# Autodesk Inventor assembly: LR_06
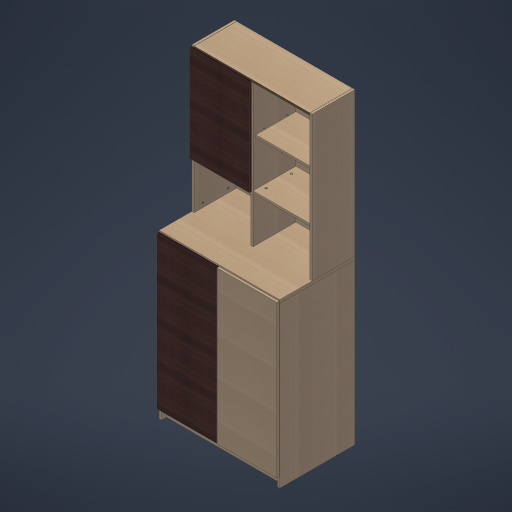
[picture p0: Inventor's stored thumbnail of the model, 512x512]
Saved by Autodesk Inventor 2024.3 (Build 283343000, 343)
## iProperties
Created: 2013-04-02
Part Number: LR_06
Document SubType Name: Assembly
Designer: User
Description: Side Shelf
Author: User
## Documents named in this file (30)
- C:\W4INV 2024 Design\PROJECTS\Living Room\Side Cabinet\LR_06.iam
- C:\W4INV 2024 Design\PROJECTS\Samples\Living Room\Side Cabinet\LR_0604.ipt
- C:\W4INV 2024 Design\PROJECTS\Samples\Living Room\Side Cabinet\LR_0611.ipt
- C:\W4INV 2024 Design\PROJECTS\Samples\Living Room\Side Cabinet\LR_0605.ipt
- C:\W4INV 2024 Design\PROJECTS\Samples\Living Room\Side Cabinet\LR_0608.ipt
- C:\W4INV 2024 Design\PROJECTS\Samples\Living Room\Side Cabinet\LR_0613.ipt
- C:\W4INV 2024 Design\PROJECTS\Samples\Living Room\Side Cabinet\LR_0607.ipt
- C:\W4INV 2024 Design\PROJECTS\Samples\Living Room\Side Cabinet\LR_0612.ipt
- C:\W4INV 2024 Design\PROJECTS\Samples\Living Room\Side Cabinet\LR_0606.ipt
- C:\W4INV 2024 Design\PROJECTS\Samples\Living Room\Side Cabinet\LR_0617.ipt
- C:\W4INV 2024 Design\PROJECTS\Samples\Living Room\Side Cabinet\LR_0616.ipt
- C:\W4INV 2024 Design\PROJECTS\Samples\Living Room\Side Cabinet\LR_0610.ipt
- C:\W4INV 2024 Design\PROJECTS\Samples\Living Room\Side Cabinet\LR_0609.ipt
- C:\W4INV 2024 Design\PROJECTS\Samples\Living Room\Side Cabinet\LR_0614.ipt
- C:\W4INV 2024 Design\PROJECTS\Samples\Living Room\Side Cabinet\LR_0619.ipt
- C:\W4INV 2024 Design\PROJECTS\Samples\Living Room\Side Cabinet\LR_0602.ipt
- C:\W4INV 2024 Design\PROJECTS\Samples\Living Room\Side Cabinet\LR_0618.ipt
- C:\W4INV 2024 Design\PROJECTS\Samples\Living Room\Side Cabinet\LR_0615.ipt
- C:\W4INV 2024 Design\PROJECTS\Samples\Living Room\Side Cabinet\SkeletonLR_0600.ipt
- C:\W4INV 2024 Design\PROJECTS\Samples\Living Room\Side Cabinet\LR_0601.ipt
- C:\W4INV 2024 Design\PROJECTS\Samples\Living Room\Side Cabinet\LR_0603.ipt
- C:\W4INV 2024 Design\_LIBRARY\Hinges\CONCEALED HINGE\Full Overlay Hinge Wood Screw Cup Wood Screw T18.iam
- C:\W4INV 2024 Design\_LIBRARY\Holders\Shelf holder D5\Shelf support D5 L16 HOL 3 CAP ON.ipt
- C:\W4INV 2024 Design\_LIBRARY\Fixed joints\Minifix joint\MINIFIX D15 v2\Minifix D15 & Dowel L34 & Cap D15 PB T18 LH.ipt
- C:\W4INV 2024 Design\_LIBRARY\Fixed joints\Minifix joint\MINIFIX D15 v2\Minifix D15 & Dowel L34 & Cap D15 PB T18 RH.ipt
- C:\W4INV 2024 Design\_LIBRARY\Supports and legs\Supports\ADJUSTABLE SUPPORT\Support M6 H27 D18 with Bushing SB T18.ipt
- C:\W4INV 2023 Design\LIBRARY\Hinges\CONCEALED HINGE.iam
- C:\W4INV 2023 Design\LIBRARY\Holders\Shelf holder D5.ipt
- C:\W4INV 2023 Design\LIBRARY\Supports and legs\Supports\ADJUSTABLE SUPPORT.ipt
- C:\W4INV 2023 Design\LIBRARY\Fixed joints\Minifix joint\MINIFIX D15 v2.ipt
## Components (84 placed, 24 different names)
1. LR_0604-Top Partition:1 — Mate:98, Mate:100, Mate:102, Mate:104, Mate:106, Mate:108, Mate:114, Mate:118, Mate:138, Mate:140, Mate:142, Mate:144
2. LR_0611-Left Side:1 — Flush:7, Flush:8, Mate:32, Flush:107, Mate:34, Flush:108, Mate:44, Mate:50, Flush:113, Mate:84, Mate:86, Flush:115, Mate:88, Mate:90, Mate:122, Mate:126, Flush:143, Flush:145
3. LR_0605-Right Side:1 — Mate:40, Flush:111, Mate:42, Flush:112, Flush:114, Flush:116, Mate:124, Mate:128, Flush:144, Flush:146
4. LR_0608-Bottom:1 — Mate:116, Mate:120, Flush:135, Flush:136, Flush:137, Flush:138
5. LR_0613-Left Door:1 — Flush:3, Flush:4
6. LR_0607-Right Door:1
7. LR_0612-Left Upper Side:1 — Flush:5, Flush:6, Mate:36, Flush:109, Mate:38, Flush:110, Mate:56, Mate:68, Flush:123, Flush:126, Mate:130, Mate:134, Mate:146, Mate:154
8. LR_0606-Right Upper Side:1 — Mate:65, Mate:77, Flush:124, Flush:127, Mate:132, Mate:136, Mate:152, Mate:160
9. LR_0617-Top:1 — Mate:110, Mate:112, Flush:139, Flush:140, Flush:141, Flush:142
10. LR_0616-Vertical Upper Partition:1 — Mate:59, Mate:62, Mate:71, Mate:74, Flush:125, Flush:128, Flush:129, Flush:130, Mate:148, Mate:150, Mate:156, Mate:158
11. LR_0610-Left Horizontal Partition:1 — Flush:147, Flush:148, Flush:149, Flush:150, Flush:151, Flush:152, Flush:153, Flush:154
12. LR_0609-Right Horizontal Partition:1
13. LR_0619-Upper Door:1 — Flush:1, Flush:2
14. LR_0602-Lower Back:1
15. LR_0618-Top Back:1
16. LR_0615-Plynth:1
17. LR_0603-Lover Vertical Partition:1 — Mate:47, Mate:53, Flush:131, Flush:132, Flush:133, Flush:134
18. Full Overlay Hinge Wood Screw Cup Wood Screw T18:1 [sub-assembly] — Mate:31, Mate:32, Flush:107
19. Full Overlay Hinge Wood Screw Cup Wood Screw T18:2 [sub-assembly] — Mate:33, Mate:34, Flush:108
20. Full Overlay Hinge Wood Screw Cup Wood Screw T18:3 [sub-assembly] — Mate:35, Mate:36, Flush:109
21. Full Overlay Hinge Wood Screw Cup Wood Screw T18:4 [sub-assembly] — Mate:37, Mate:38, Flush:110
22. Full Overlay Hinge Wood Screw Cup Wood Screw T18:5 [sub-assembly] — Mate:39, Mate:40, Flush:111
23. Full Overlay Hinge Wood Screw Cup Wood Screw T18:6 [sub-assembly] — Mate:41, Mate:42, Flush:112
24. Shelf support D5 L16 HOL 3 CAP ON:13 — Mate:56, Mate:57, Mate:79
25. Shelf support D5 L16 HOL 3 CAP ON:14 — Mate:59, Mate:60, Mate:80
26. Shelf support D5 L16 HOL 3 CAP ON:15 — Mate:62, Mate:63, Mate:81
27. Shelf support D5 L16 HOL 3 CAP ON:16 — Mate:65, Mate:66, Mate:82
28. Shelf support D5 L16 HOL 3 CAP ON:17 — Mate:67, Mate:68, Mate:69
29. Shelf support D5 L16 HOL 3 CAP ON:18 — Mate:70, Mate:71, Mate:72
30. Shelf support D5 L16 HOL 3 CAP ON:19 — Mate:73, Mate:74, Mate:75
31. Shelf support D5 L16 HOL 3 CAP ON:20 — Mate:76, Mate:77, Mate:78
32. Support M6 H27 D18 with Bushing SB T18:6 — Mate:83, Flush:113, Mate:84
33. Support M6 H27 D18 with Bushing SB T18:7 — Mate:85, Flush:114, Mate:86
34. Support M6 H27 D18 with Bushing SB T18:8 — Mate:87, Flush:115, Mate:88
35. Support M6 H27 D18 with Bushing SB T18:9 — Mate:89, Flush:116, Mate:90
36. Minifix D15 & Dowel L34 & Cap D15 PB T18 RH:7 — Mate:97, Flush:123, Mate:98
37. Minifix D15 & Dowel L34 & Cap D15 PB T18 LH:8 — Mate:99, Flush:124, Mate:100
38. Minifix D15 & Dowel L34 & Cap D15 PB T18 LH:9 — Mate:101, Flush:125, Mate:102
39. Minifix D15 & Dowel L34 & Cap D15 PB T18 LH:10 — Mate:103, Flush:126, Mate:104
40. Minifix D15 & Dowel L34 & Cap D15 PB T18 RH:11 — Mate:105, Flush:127, Mate:106
41. Minifix D15 & Dowel L34 & Cap D15 PB T18 RH:12 — Mate:107, Flush:128, Mate:108
42. Minifix D15 & Dowel L34 & Cap D15 PB T18 RH:13 — Mate:109, Mate:110, Flush:129
43. Minifix D15 & Dowel L34 & Cap D15 PB T18 LH:14 — Mate:111, Mate:112, Flush:130
44. Minifix D15 & Dowel L34 & Cap D15 PB T18 RH:15 — Mate:113, Mate:114, Flush:131
45. Minifix D15 & Dowel L34 & Cap D15 PB T18 LH:16 — Mate:115, Mate:116, Flush:132
46. Minifix D15 & Dowel L34 & Cap D15 PB T18 LH:17 — Mate:117, Mate:118, Flush:133
47. Minifix D15 & Dowel L34 & Cap D15 PB T18 RH:18 — Mate:119, Mate:120, Flush:134
48. Minifix D15 & Dowel L34 & Cap D15 PB T18 LH:19 — Mate:121, Mate:122, Flush:135
49. Minifix D15 & Dowel L34 & Cap D15 PB T18 RH:20 — Mate:123, Mate:124, Flush:136
50. Minifix D15 & Dowel L34 & Cap D15 PB T18 RH:21 — Mate:125, Mate:126, Flush:137
51. Minifix D15 & Dowel L34 & Cap D15 PB T18 LH:22 — Mate:127, Mate:128, Flush:138
52. Minifix D15 & Dowel L34 & Cap D15 PB T18 RH:23 — Mate:129, Mate:130, Flush:139
53. Minifix D15 & Dowel L34 & Cap D15 PB T18 LH:24 — Mate:131, Mate:132, Flush:140
54. Minifix D15 & Dowel L34 & Cap D15 PB T18 LH:25 — Mate:133, Mate:134, Flush:141
55. Minifix D15 & Dowel L34 & Cap D15 PB T18 RH:26 — Mate:135, Mate:136, Flush:142
56. Minifix D15 & Dowel L34 & Cap D15 PB T18 LH:27 — Mate:137, Flush:143, Mate:138
57. Minifix D15 & Dowel L34 & Cap D15 PB T18 RH:28 — Mate:139, Flush:144, Mate:140
58. Minifix D15 & Dowel L34 & Cap D15 PB T18 RH:29 — Mate:141, Flush:145, Mate:142
59. Minifix D15 & Dowel L34 & Cap D15 PB T18 LH:30 — Mate:143, Flush:146, Mate:144
60. Minifix D15 & Dowel L34 & Cap D15 PB T18 LH:31 — Mate:145, Mate:146, Flush:147
61. Minifix D15 & Dowel L34 & Cap D15 PB T18 RH:32 — Mate:147, Mate:148, Flush:148
62. Minifix D15 & Dowel L34 & Cap D15 PB T18 LH:33 — Mate:149, Mate:150, Flush:149
63. Minifix D15 & Dowel L34 & Cap D15 PB T18 RH:34 — Mate:151, Mate:152, Flush:150
64. Minifix D15 & Dowel L34 & Cap D15 PB T18 RH:35 — Mate:153, Mate:154, Flush:151
65. Minifix D15 & Dowel L34 & Cap D15 PB T18 RH:36 — Mate:155, Mate:156, Flush:152
66. Minifix D15 & Dowel L34 & Cap D15 PB T18 LH:37 — Mate:157, Mate:158, Flush:153
67. Minifix D15 & Dowel L34 & Cap D15 PB T18 LH:38 — Mate:159, Mate:160, Flush:154
68. LR_0614-Shelve:1 — Mate:57, Mate:60, Mate:63, Mate:66, Mate:69, Mate:72, Mate:75, Mate:78
69. LR_0614-Shelve:2
70. LR_0601-Lower Shelve:1 — Mate:45, Mate:48, Mate:51, Mate:54
71. Shelf support D5 L16 HOL 3 CAP ON:1 — Mate:43, Mate:44, Mate:45
72. Shelf support D5 L16 HOL 3 CAP ON:3 — Mate:49, Mate:50, Mate:51
73. Shelf support D5 L16 HOL 3 CAP ON:4 — Mate:52, Mate:53, Mate:54
74. Shelf support D5 L16 HOL 3 CAP ON:2 — Mate:46, Mate:47, Mate:48
75. LR_0601-Lower Shelve:2
76. Shelf support D5 L16 HOL 3 CAP ON:5
77. Shelf support D5 L16 HOL 3 CAP ON:7
78. Shelf support D5 L16 HOL 3 CAP ON:9
79. Shelf support D5 L16 HOL 3 CAP ON:11
80. LR_0601-Lower Shelve:3
81. Shelf support D5 L16 HOL 3 CAP ON:6
82. Shelf support D5 L16 HOL 3 CAP ON:8
83. Shelf support D5 L16 HOL 3 CAP ON:10
84. Shelf support D5 L16 HOL 3 CAP ON:12
## Component patterns: (2 elements, first: LR_0614-Shelve:1), (3 elements, first: LR_0601-Lower Shelve:1 + Shelf support D5 L16 HOL 3 CAP ON:1 + Shelf support D5 L16 HOL 3 CAP ON:3 + Shelf support D5 L16 HOL 3 CAP ON:4 + Shelf support D5 L16 HOL 3 CAP ON:2)
## Relationships (172: Mate 120, Flush 52)
- Flush:1 (-100 mm): LR_0619-Upper Door:1
- Flush:2 (-100 mm): LR_0619-Upper Door:1
- Flush:3 (-100 mm): LR_0613-Left Door:1
- Flush:4 (-100 mm): LR_0613-Left Door:1
- Flush:5 (-70 mm): LR_0612-Left Upper Side:1
- Flush:6 (-70 mm): LR_0612-Left Upper Side:1
- Flush:7 (-134 mm): LR_0611-Left Side:1
- Flush:8 (-80 mm): LR_0611-Left Side:1
- Flush:45 (-16 mm)
- Flush:46 (-16 mm)
- Mate:31: Full Overlay Hinge Wood Screw Cup Wood Screw T18:1
- Mate:32: LR_0611-Left Side:1 ↔ Full Overlay Hinge Wood Screw Cup Wood Screw T18:1
- Flush:107: LR_0611-Left Side:1 ↔ Full Overlay Hinge Wood Screw Cup Wood Screw T18:1
- Mate:33: Full Overlay Hinge Wood Screw Cup Wood Screw T18:2
- Mate:34: LR_0611-Left Side:1 ↔ Full Overlay Hinge Wood Screw Cup Wood Screw T18:2
- Flush:108: LR_0611-Left Side:1 ↔ Full Overlay Hinge Wood Screw Cup Wood Screw T18:2
- Mate:35: Full Overlay Hinge Wood Screw Cup Wood Screw T18:3
- Mate:36: LR_0612-Left Upper Side:1 ↔ Full Overlay Hinge Wood Screw Cup Wood Screw T18:3
- Flush:109: LR_0612-Left Upper Side:1 ↔ Full Overlay Hinge Wood Screw Cup Wood Screw T18:3
- Mate:37: Full Overlay Hinge Wood Screw Cup Wood Screw T18:4
- Mate:38: LR_0612-Left Upper Side:1 ↔ Full Overlay Hinge Wood Screw Cup Wood Screw T18:4
- Flush:110: LR_0612-Left Upper Side:1 ↔ Full Overlay Hinge Wood Screw Cup Wood Screw T18:4
- Mate:39: Full Overlay Hinge Wood Screw Cup Wood Screw T18:5
- Mate:40: LR_0605-Right Side:1 ↔ Full Overlay Hinge Wood Screw Cup Wood Screw T18:5
- Flush:111: LR_0605-Right Side:1 ↔ Full Overlay Hinge Wood Screw Cup Wood Screw T18:5
- Mate:41: Full Overlay Hinge Wood Screw Cup Wood Screw T18:6
- Mate:42: LR_0605-Right Side:1 ↔ Full Overlay Hinge Wood Screw Cup Wood Screw T18:6
- Flush:112: LR_0605-Right Side:1 ↔ Full Overlay Hinge Wood Screw Cup Wood Screw T18:6
- Mate:43: Shelf support D5 L16 HOL 3 CAP ON:1
- Mate:44: LR_0611-Left Side:1 ↔ Shelf support D5 L16 HOL 3 CAP ON:1
- Mate:45 (2.5 mm): LR_0601-Lower Shelve:1 ↔ Shelf support D5 L16 HOL 3 CAP ON:1
- Mate:46: Shelf support D5 L16 HOL 3 CAP ON:2
- Mate:47: LR_0603-Lover Vertical Partition:1 ↔ Shelf support D5 L16 HOL 3 CAP ON:2
- Mate:48 (2.5 mm): LR_0601-Lower Shelve:1 ↔ Shelf support D5 L16 HOL 3 CAP ON:2
- Mate:49: Shelf support D5 L16 HOL 3 CAP ON:3
- Mate:50: LR_0611-Left Side:1 ↔ Shelf support D5 L16 HOL 3 CAP ON:3
- Mate:51 (2.5 mm): LR_0601-Lower Shelve:1 ↔ Shelf support D5 L16 HOL 3 CAP ON:3
- Mate:52: Shelf support D5 L16 HOL 3 CAP ON:4
- Mate:53: LR_0603-Lover Vertical Partition:1 ↔ Shelf support D5 L16 HOL 3 CAP ON:4
- Mate:54 (2.5 mm): LR_0601-Lower Shelve:1 ↔ Shelf support D5 L16 HOL 3 CAP ON:4
- Mate:56: LR_0612-Left Upper Side:1 ↔ Shelf support D5 L16 HOL 3 CAP ON:13
- Mate:57 (2.5 mm): Shelf support D5 L16 HOL 3 CAP ON:13 ↔ LR_0614-Shelve:1
- Mate:59: LR_0616-Vertical Upper Partition:1 ↔ Shelf support D5 L16 HOL 3 CAP ON:14
- Mate:60 (2.5 mm): Shelf support D5 L16 HOL 3 CAP ON:14 ↔ LR_0614-Shelve:1
- Mate:62: LR_0616-Vertical Upper Partition:1 ↔ Shelf support D5 L16 HOL 3 CAP ON:15
- Mate:63 (2.5 mm): Shelf support D5 L16 HOL 3 CAP ON:15 ↔ LR_0614-Shelve:1
- Mate:65: LR_0606-Right Upper Side:1 ↔ Shelf support D5 L16 HOL 3 CAP ON:16
- Mate:66 (2.5 mm): Shelf support D5 L16 HOL 3 CAP ON:16 ↔ LR_0614-Shelve:1
- Mate:67: Shelf support D5 L16 HOL 3 CAP ON:17
- Mate:68: LR_0612-Left Upper Side:1 ↔ Shelf support D5 L16 HOL 3 CAP ON:17
- Mate:69 (2.5 mm): Shelf support D5 L16 HOL 3 CAP ON:17 ↔ LR_0614-Shelve:1
- Mate:70: Shelf support D5 L16 HOL 3 CAP ON:18
- Mate:71: LR_0616-Vertical Upper Partition:1 ↔ Shelf support D5 L16 HOL 3 CAP ON:18
- Mate:72 (2.5 mm): Shelf support D5 L16 HOL 3 CAP ON:18 ↔ LR_0614-Shelve:1
- Mate:73: Shelf support D5 L16 HOL 3 CAP ON:19
- Mate:74: LR_0616-Vertical Upper Partition:1 ↔ Shelf support D5 L16 HOL 3 CAP ON:19
- Mate:75 (2.5 mm): Shelf support D5 L16 HOL 3 CAP ON:19 ↔ LR_0614-Shelve:1
- Mate:76: Shelf support D5 L16 HOL 3 CAP ON:20
- Mate:77: LR_0606-Right Upper Side:1 ↔ Shelf support D5 L16 HOL 3 CAP ON:20
- Mate:78 (2.5 mm): Shelf support D5 L16 HOL 3 CAP ON:20 ↔ LR_0614-Shelve:1
- Mate:79: Shelf support D5 L16 HOL 3 CAP ON:13
- Mate:80: Shelf support D5 L16 HOL 3 CAP ON:14
- Mate:81: Shelf support D5 L16 HOL 3 CAP ON:15
- Mate:82: Shelf support D5 L16 HOL 3 CAP ON:16
- Mate:83: Support M6 H27 D18 with Bushing SB T18:6
- Flush:113 (9 mm): LR_0611-Left Side:1 ↔ Support M6 H27 D18 with Bushing SB T18:6
- Mate:84 (17.5 mm): LR_0611-Left Side:1 ↔ Support M6 H27 D18 with Bushing SB T18:6
- Mate:85: Support M6 H27 D18 with Bushing SB T18:7
- Flush:114 (9 mm): LR_0605-Right Side:1 ↔ Support M6 H27 D18 with Bushing SB T18:7
- Mate:86 (17.5 mm): LR_0611-Left Side:1 ↔ Support M6 H27 D18 with Bushing SB T18:7
- Mate:87: Support M6 H27 D18 with Bushing SB T18:8
- Flush:115 (9 mm): LR_0611-Left Side:1 ↔ Support M6 H27 D18 with Bushing SB T18:8
- Mate:88 (17.5 mm): LR_0611-Left Side:1 ↔ Support M6 H27 D18 with Bushing SB T18:8
- Mate:89: Support M6 H27 D18 with Bushing SB T18:9
- Flush:116 (9 mm): LR_0605-Right Side:1 ↔ Support M6 H27 D18 with Bushing SB T18:9
- Mate:90 (17.5 mm): LR_0611-Left Side:1 ↔ Support M6 H27 D18 with Bushing SB T18:9
- Mate:97: Minifix D15 & Dowel L34 & Cap D15 PB T18 RH:7
- Flush:123 (18 mm): LR_0612-Left Upper Side:1 ↔ Minifix D15 & Dowel L34 & Cap D15 PB T18 RH:7
- Mate:98: LR_0604-Top Partition:1 ↔ Minifix D15 & Dowel L34 & Cap D15 PB T18 RH:7
- Mate:99: Minifix D15 & Dowel L34 & Cap D15 PB T18 LH:8
- Flush:124 (18 mm): LR_0606-Right Upper Side:1 ↔ Minifix D15 & Dowel L34 & Cap D15 PB T18 LH:8
- Mate:100: LR_0604-Top Partition:1 ↔ Minifix D15 & Dowel L34 & Cap D15 PB T18 LH:8
- Mate:101: Minifix D15 & Dowel L34 & Cap D15 PB T18 LH:9
- Flush:125 (18 mm): LR_0616-Vertical Upper Partition:1 ↔ Minifix D15 & Dowel L34 & Cap D15 PB T18 LH:9
- Mate:102: LR_0604-Top Partition:1 ↔ Minifix D15 & Dowel L34 & Cap D15 PB T18 LH:9
- Mate:103: Minifix D15 & Dowel L34 & Cap D15 PB T18 LH:10
- Flush:126 (18 mm): LR_0612-Left Upper Side:1 ↔ Minifix D15 & Dowel L34 & Cap D15 PB T18 LH:10
- Mate:104: LR_0604-Top Partition:1 ↔ Minifix D15 & Dowel L34 & Cap D15 PB T18 LH:10
- Mate:105: Minifix D15 & Dowel L34 & Cap D15 PB T18 RH:11
- Flush:127 (18 mm): LR_0606-Right Upper Side:1 ↔ Minifix D15 & Dowel L34 & Cap D15 PB T18 RH:11
- Mate:106: LR_0604-Top Partition:1 ↔ Minifix D15 & Dowel L34 & Cap D15 PB T18 RH:11
- Mate:107: Minifix D15 & Dowel L34 & Cap D15 PB T18 RH:12
- Flush:128 (18 mm): LR_0616-Vertical Upper Partition:1 ↔ Minifix D15 & Dowel L34 & Cap D15 PB T18 RH:12
- Mate:108: LR_0604-Top Partition:1 ↔ Minifix D15 & Dowel L34 & Cap D15 PB T18 RH:12
- Mate:109: Minifix D15 & Dowel L34 & Cap D15 PB T18 RH:13
- Mate:110: LR_0617-Top:1 ↔ Minifix D15 & Dowel L34 & Cap D15 PB T18 RH:13
- Flush:129 (18 mm): LR_0616-Vertical Upper Partition:1 ↔ Minifix D15 & Dowel L34 & Cap D15 PB T18 RH:13
- Mate:111: Minifix D15 & Dowel L34 & Cap D15 PB T18 LH:14
- Mate:112: LR_0617-Top:1 ↔ Minifix D15 & Dowel L34 & Cap D15 PB T18 LH:14
- Flush:130 (18 mm): LR_0616-Vertical Upper Partition:1 ↔ Minifix D15 & Dowel L34 & Cap D15 PB T18 LH:14
- Mate:113: Minifix D15 & Dowel L34 & Cap D15 PB T18 RH:15
- Mate:114: LR_0604-Top Partition:1 ↔ Minifix D15 & Dowel L34 & Cap D15 PB T18 RH:15
- Flush:131 (18 mm): LR_0603-Lover Vertical Partition:1 ↔ Minifix D15 & Dowel L34 & Cap D15 PB T18 RH:15
- Mate:115: Minifix D15 & Dowel L34 & Cap D15 PB T18 LH:16
- Mate:116: LR_0608-Bottom:1 ↔ Minifix D15 & Dowel L34 & Cap D15 PB T18 LH:16
- Flush:132 (18 mm): LR_0603-Lover Vertical Partition:1 ↔ Minifix D15 & Dowel L34 & Cap D15 PB T18 LH:16
- Mate:117: Minifix D15 & Dowel L34 & Cap D15 PB T18 LH:17
- Mate:118: LR_0604-Top Partition:1 ↔ Minifix D15 & Dowel L34 & Cap D15 PB T18 LH:17
- Flush:133 (18 mm): LR_0603-Lover Vertical Partition:1 ↔ Minifix D15 & Dowel L34 & Cap D15 PB T18 LH:17
- Mate:119: Minifix D15 & Dowel L34 & Cap D15 PB T18 RH:18
- Mate:120: LR_0608-Bottom:1 ↔ Minifix D15 & Dowel L34 & Cap D15 PB T18 RH:18
- Flush:134 (18 mm): LR_0603-Lover Vertical Partition:1 ↔ Minifix D15 & Dowel L34 & Cap D15 PB T18 RH:18
- Mate:121: Minifix D15 & Dowel L34 & Cap D15 PB T18 LH:19
- Mate:122: LR_0611-Left Side:1 ↔ Minifix D15 & Dowel L34 & Cap D15 PB T18 LH:19
- Flush:135 (18 mm): LR_0608-Bottom:1 ↔ Minifix D15 & Dowel L34 & Cap D15 PB T18 LH:19
- Mate:123: Minifix D15 & Dowel L34 & Cap D15 PB T18 RH:20
- Mate:124: LR_0605-Right Side:1 ↔ Minifix D15 & Dowel L34 & Cap D15 PB T18 RH:20
- Flush:136 (18 mm): LR_0608-Bottom:1 ↔ Minifix D15 & Dowel L34 & Cap D15 PB T18 RH:20
- Mate:125: Minifix D15 & Dowel L34 & Cap D15 PB T18 RH:21
- Mate:126: LR_0611-Left Side:1 ↔ Minifix D15 & Dowel L34 & Cap D15 PB T18 RH:21
- Flush:137 (18 mm): LR_0608-Bottom:1 ↔ Minifix D15 & Dowel L34 & Cap D15 PB T18 RH:21
- Mate:127: Minifix D15 & Dowel L34 & Cap D15 PB T18 LH:22
- Mate:128: LR_0605-Right Side:1 ↔ Minifix D15 & Dowel L34 & Cap D15 PB T18 LH:22
- Flush:138 (18 mm): LR_0608-Bottom:1 ↔ Minifix D15 & Dowel L34 & Cap D15 PB T18 LH:22
- Mate:129: Minifix D15 & Dowel L34 & Cap D15 PB T18 RH:23
- Mate:130: LR_0612-Left Upper Side:1 ↔ Minifix D15 & Dowel L34 & Cap D15 PB T18 RH:23
- Flush:139 (18 mm): LR_0617-Top:1 ↔ Minifix D15 & Dowel L34 & Cap D15 PB T18 RH:23
- Mate:131: Minifix D15 & Dowel L34 & Cap D15 PB T18 LH:24
- Mate:132: LR_0606-Right Upper Side:1 ↔ Minifix D15 & Dowel L34 & Cap D15 PB T18 LH:24
- Flush:140 (18 mm): LR_0617-Top:1 ↔ Minifix D15 & Dowel L34 & Cap D15 PB T18 LH:24
- Mate:133: Minifix D15 & Dowel L34 & Cap D15 PB T18 LH:25
- Mate:134: LR_0612-Left Upper Side:1 ↔ Minifix D15 & Dowel L34 & Cap D15 PB T18 LH:25
- Flush:141 (18 mm): LR_0617-Top:1 ↔ Minifix D15 & Dowel L34 & Cap D15 PB T18 LH:25
- Mate:135: Minifix D15 & Dowel L34 & Cap D15 PB T18 RH:26
- Mate:136: LR_0606-Right Upper Side:1 ↔ Minifix D15 & Dowel L34 & Cap D15 PB T18 RH:26
- Flush:142 (18 mm): LR_0617-Top:1 ↔ Minifix D15 & Dowel L34 & Cap D15 PB T18 RH:26
- Mate:137: Minifix D15 & Dowel L34 & Cap D15 PB T18 LH:27
- Flush:143 (18 mm): LR_0611-Left Side:1 ↔ Minifix D15 & Dowel L34 & Cap D15 PB T18 LH:27
- Mate:138: LR_0604-Top Partition:1 ↔ Minifix D15 & Dowel L34 & Cap D15 PB T18 LH:27
- Mate:139: Minifix D15 & Dowel L34 & Cap D15 PB T18 RH:28
- Flush:144 (18 mm): LR_0605-Right Side:1 ↔ Minifix D15 & Dowel L34 & Cap D15 PB T18 RH:28
- Mate:140: LR_0604-Top Partition:1 ↔ Minifix D15 & Dowel L34 & Cap D15 PB T18 RH:28
- Mate:141: Minifix D15 & Dowel L34 & Cap D15 PB T18 RH:29
- Flush:145 (18 mm): LR_0611-Left Side:1 ↔ Minifix D15 & Dowel L34 & Cap D15 PB T18 RH:29
- Mate:142: LR_0604-Top Partition:1 ↔ Minifix D15 & Dowel L34 & Cap D15 PB T18 RH:29
- Mate:143: Minifix D15 & Dowel L34 & Cap D15 PB T18 LH:30
- Flush:146 (18 mm): LR_0605-Right Side:1 ↔ Minifix D15 & Dowel L34 & Cap D15 PB T18 LH:30
- Mate:144: LR_0604-Top Partition:1 ↔ Minifix D15 & Dowel L34 & Cap D15 PB T18 LH:30
- Mate:145: Minifix D15 & Dowel L34 & Cap D15 PB T18 LH:31
- Mate:146: LR_0612-Left Upper Side:1 ↔ Minifix D15 & Dowel L34 & Cap D15 PB T18 LH:31
- Flush:147 (18 mm): LR_0610-Left Horizontal Partition:1 ↔ Minifix D15 & Dowel L34 & Cap D15 PB T18 LH:31
- Mate:147: Minifix D15 & Dowel L34 & Cap D15 PB T18 RH:32
- Mate:148: LR_0616-Vertical Upper Partition:1 ↔ Minifix D15 & Dowel L34 & Cap D15 PB T18 RH:32
- Flush:148 (18 mm): LR_0610-Left Horizontal Partition:1 ↔ Minifix D15 & Dowel L34 & Cap D15 PB T18 RH:32
- Mate:149: Minifix D15 & Dowel L34 & Cap D15 PB T18 LH:33
- Mate:150: LR_0616-Vertical Upper Partition:1 ↔ Minifix D15 & Dowel L34 & Cap D15 PB T18 LH:33
- Flush:149 (18 mm): LR_0610-Left Horizontal Partition:1 ↔ Minifix D15 & Dowel L34 & Cap D15 PB T18 LH:33
- Mate:151: Minifix D15 & Dowel L34 & Cap D15 PB T18 RH:34
- Mate:152: LR_0606-Right Upper Side:1 ↔ Minifix D15 & Dowel L34 & Cap D15 PB T18 RH:34
- Flush:150 (18 mm): LR_0610-Left Horizontal Partition:1 ↔ Minifix D15 & Dowel L34 & Cap D15 PB T18 RH:34
- Mate:153: Minifix D15 & Dowel L34 & Cap D15 PB T18 RH:35
- Mate:154: LR_0612-Left Upper Side:1 ↔ Minifix D15 & Dowel L34 & Cap D15 PB T18 RH:35
- Flush:151 (18 mm): LR_0610-Left Horizontal Partition:1 ↔ Minifix D15 & Dowel L34 & Cap D15 PB T18 RH:35
- Mate:155: Minifix D15 & Dowel L34 & Cap D15 PB T18 RH:36
- Mate:156: LR_0616-Vertical Upper Partition:1 ↔ Minifix D15 & Dowel L34 & Cap D15 PB T18 RH:36
- Flush:152 (18 mm): LR_0610-Left Horizontal Partition:1 ↔ Minifix D15 & Dowel L34 & Cap D15 PB T18 RH:36
- Mate:157: Minifix D15 & Dowel L34 & Cap D15 PB T18 LH:37
- Mate:158: LR_0616-Vertical Upper Partition:1 ↔ Minifix D15 & Dowel L34 & Cap D15 PB T18 LH:37
- Flush:153 (18 mm): LR_0610-Left Horizontal Partition:1 ↔ Minifix D15 & Dowel L34 & Cap D15 PB T18 LH:37
- Mate:159: Minifix D15 & Dowel L34 & Cap D15 PB T18 LH:38
- Mate:160: LR_0606-Right Upper Side:1 ↔ Minifix D15 & Dowel L34 & Cap D15 PB T18 LH:38
- Flush:154 (18 mm): LR_0610-Left Horizontal Partition:1 ↔ Minifix D15 & Dowel L34 & Cap D15 PB T18 LH:38
## Named parameters: Tarp_Pertvaru = 470.36797 mm
